# Autodesk Inventor assembly: Редуктор в сборе
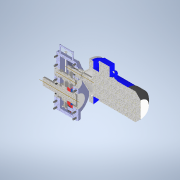
[picture p0: Inventor's stored thumbnail of the model, 180x180]
Saved by Autodesk Inventor 2021 (Build 250183000, 183)
## iProperties
Created: 2023-03-03
Part Number: Редуктор в сборе
Document SubType Name: Assembly
Designer: gdevc
Mass: 20906 g
Surface Area: 13580.9 cm^2
Volume: 12356.7 cm^3
Density: 1.69188 g/cm^3
Author: gdevc
## Documents named in this file (26)
- C:\Users\gdevc\OneDrive\Рабочий стол\Курсач\DetaliMashine\Новая папка\Редуктор в сборе.iam
- C:\Users\gdevc\OneDrive\Рабочий стол\Курсач\DetaliMashine\Новая папка\Вал_промежуточный.ipt
- C:\Users\gdevc\OneDrive\Рабочий стол\Курсач\DetaliMashine\Новая папка\Редуктор в сборе\Мастер проектирования\Цилиндрическое зубчатое зацепление1.iam
- C:\Users\gdevc\OneDrive\Рабочий стол\Курсач\DetaliMashine\Новая папка\Колесо быстроходное.ipt
- C:\Users\gdevc\OneDrive\Рабочий стол\Курсач\DetaliMashine\Новая папка\Редуктор в сборе\Мастер проектирования\Цилиндрическое зубчатое зацепление2.iam
- C:\Users\gdevc\OneDrive\Рабочий стол\Курсач\DetaliMashine\Новая папка\Вал_тихоходный.ipt
- C:\Users\gdevc\OneDrive\Рабочий стол\Курсач\DetaliMashine\Новая папка\Редуктор в сборе\Мастер проектирования\Цилиндрическое зубчатое зацепление3.iam
- C:\Users\gdevc\OneDrive\Рабочий стол\Курсач\DetaliMashine\Новая папка\Валл быстроходный.ipt
- C:\Users\gdevc\OneDrive\Рабочий стол\Курсач\DetaliMashine\Новая папка\Редуктор в сборе\Мастер проектирования\Цилиндрическое зубчатое зацепление4.iam
- C:\Users\gdevc\OneDrive\Рабочий стол\Курсач\DetaliMashine\Новая папка\Крышка тих_выход.ipt
- C:\Users\gdevc\OneDrive\Рабочий стол\Курсач\DetaliMashine\Новая папка\Крышка, тихая.ipt
- C:\Users\gdevc\OneDrive\Рабочий стол\Курсач\DetaliMashine\Новая папка\Крышка_пром.ipt
- C:\Users\gdevc\OneDrive\Рабочий стол\Курсач\DetaliMashine\Новая папка\Корпус.v.2.0.iam
- C:\Users\gdevc\OneDrive\Рабочий стол\Курсач\DetaliMashine\Новая папка\Манжет 1-30x47x7 ГОСТ 8752-79.ipt
- C:\Users\gdevc\OneDrive\Рабочий стол\Курсач\DetaliMashine\Новая папка\Крышка_быстроходного.ipt
- C:\Users\gdevc\OneDrive\Рабочий стол\Курсач\DetaliMashine\Новая папка\Подшипник 210 ГОСТ 8338-75.ipt
- C:\Users\gdevc\OneDrive\Рабочий стол\Курсач\DetaliMashine\Новая папка\Подшипник 205 ГОСТ 8338-75.ipt
- C:\Users\gdevc\OneDrive\Рабочий стол\Курсач\DetaliMashine\Новая папка\Манжет 2-50x65x8 ГОСТ 8752-79.ipt
- C:\Users\gdevc\OneDrive\Рабочий стол\Курсач\DetaliMashine\Новая папка\Болт M10×35 ГОСТ Р 50793-95.ipt
- C:\Users\gdevc\OneDrive\Рабочий стол\Курсач\DetaliMashine\Новая папка\Промежуточное колесо резина.ipt
- C:\Users\gdevc\OneDrive\Рабочий стол\Курсач\DetaliMashine\Новая папка\Редуктор в сборе\Мастер проектирования\Цилиндрическое зубчатое зацепление5.iam
- C:\Users\gdevc\OneDrive\Рабочий стол\Курсач\DetaliMashine\Новая папка\Резина конец.ipt
- C:\Users\gdevc\OneDrive\Рабочий стол\Курсач\DetaliMashine\Новая папка\Редуктор в сборе\Мастер проектирования\Цилиндрическое зубчатое зацепление6.iam
- C:\Users\gdevc\Downloads\Telegram Desktop\АИР100L IM2081 (2,4,6,8 пол)....ipt
- C:\Users\gdevc\OneDrive\Рабочий стол\Курсач\DetaliMashine\Новая папка\Редуктор в сборе\Мастер проектирования\Цилиндрическое зубчатое зацепление7.iam
- C:\Users\gdevc\OneDrive\Рабочий стол\Курсач\DetaliMashine\Новая папка\Шуп масло.ipt
## Components (36 placed, 19 different names)
1. Вал_промежуточный:1 — Совмещение:68, Совмещение:69, Совмещение:70
2. Цилиндрическое зубчатое зацепление:1 [sub-assembly]
3. Колесо быстроходное:1 — Заподлицо:3, Заподлицо:4, Заподлицо:7, Совмещение:69
4. Цилиндрическое зубчатое зацепление:2 [sub-assembly]
5. Вал_тихоходный:1 — Совмещение:10, Совмещение:11, Совмещение:12, Совмещение:13, Совмещение:18, Совмещение:21, Совмещение:23, Совмещение:29, Совмещение:55, Совмещение:58
6. Цилиндрическое зубчатое зацепление:3 [sub-assembly]
7. Валл быстроходный:1 — Заподлицо:3, Совмещение:32, Угол:3, Совмещение:36, Совмещение:56, Угол:4, Совмещение:67, Заподлицо:7
8. Цилиндрическое зубчатое зацепление:4 [sub-assembly]
9. Подшипник 205 ГОСТ 8338-75:1 — Совмещение:26, Совмещение:64
10. Подшипник 205 ГОСТ 8338-75:2 — Совмещение:28, Совмещение:66, Совмещение:70
11. Подшипник 210 ГОСТ 8338-75:1 — Совмещение:10, Совмещение:11
12. Подшипник 210 ГОСТ 8338-75:2 — Совмещение:12, Совмещение:13, Совмещение:30
13. Манжет 2-50x65x8 ГОСТ 8752-79:1 — Совмещение:18
14. Крышка тих_выход:1 — Совмещение:21, Совмещение:30, Совмещение:71
15. Крышка, тихая:1 — Совмещение:23, Совмещение:35
16. Крышка_пром:1 — Совмещение:26, Совмещение:63, Заподлицо:6, Совмещение:64, Совмещение:67, Совмещение:68
17. Крышка_пром:2 — Совмещение:28, Совмещение:31, Совмещение:65, Совмещение:66
18. Корпус.v.2.0:1 [sub-assembly] — Совмещение:29, Угол:2, Совмещение:31, Совмещение:34, Совмещение:35, Совмещение:37, Совмещение:38, Совмещение:39, Совмещение:40, Совмещение:41, Совмещение:42, Совмещение:43, Совмещение:44, Совмещение:45, Совмещение:46, Совмещение:47, Совмещение:48, Совмещение:49, Совмещение:50, Совмещение:51, Совмещение:52, Совмещение:53, Совмещение:54, Совмещение:59, Совмещение:61, Совмещение:62, Совмещение:63, Заподлицо:6, Совмещение:65, Совмещение:71
19. Манжет 1-30x47x7 ГОСТ 8752-79:1 — Совмещение:32, Совмещение:33
20. Крышка_быстроходного:1 — Совмещение:33, Совмещение:34, Совмещение:60
21. Болт M10×35 ГОСТ Р 50793-95:1 — Совмещение:37, Совмещение:46
22. Болт M10×35 ГОСТ Р 50793-95:2 — Совмещение:38, Совмещение:47
23. Болт M10×35 ГОСТ Р 50793-95:3 — Совмещение:39, Совмещение:49
24. Болт M10×35 ГОСТ Р 50793-95:4 — Совмещение:40, Совмещение:48
25. Болт M10×35 ГОСТ Р 50793-95:5 — Совмещение:41, Совмещение:51
26. Болт M10×35 ГОСТ Р 50793-95:6 — Совмещение:42, Совмещение:53
27. Болт M10×35 ГОСТ Р 50793-95:7 — Совмещение:43, Совмещение:50
28. Болт M10×35 ГОСТ Р 50793-95:8 — Совмещение:44, Совмещение:52
29. Болт M10×35 ГОСТ Р 50793-95:9 — Совмещение:45, Совмещение:54
30. Промежуточное колесо резина:1 — Совмещение:55, Заподлицо:4, Заподлицо:5
31. Цилиндрическое зубчатое зацепление:5 [sub-assembly]
32. Резина конец:1 — Совмещение:58, Совмещение:59, Заподлицо:5
33. Цилиндрическое зубчатое зацепление:6 [sub-assembly]
34. АИР100L IM2081 (2,4,6,8 пол)...:1 — Совмещение:56, Угол:4, Совмещение:60
35. Цилиндрическое зубчатое зацепление:7 [sub-assembly]
36. Шуп масло:1 — Совмещение:61, Совмещение:62
## Relationships (59: Mate 51, Flush 5, Angle 3)
- Совмещение:10 [Mate]: Вал_тихоходный:1 ↔ Подшипник 210 ГОСТ 8338-75:1
- Совмещение:11 [Mate]: Вал_тихоходный:1 ↔ Подшипник 210 ГОСТ 8338-75:1
- Совмещение:12 [Mate]: Вал_тихоходный:1 ↔ Подшипник 210 ГОСТ 8338-75:2
- Совмещение:13 [Mate]: Вал_тихоходный:1 ↔ Подшипник 210 ГОСТ 8338-75:2
- Совмещение:18 [Mate]: Вал_тихоходный:1 ↔ Манжет 2-50x65x8 ГОСТ 8752-79:1
- Совмещение:21 [Mate]: Вал_тихоходный:1 ↔ Крышка тих_выход:1
- Совмещение:23 [Mate]: Вал_тихоходный:1 ↔ Крышка, тихая:1
- Совмещение:26 [Mate]: Подшипник 205 ГОСТ 8338-75:1 ↔ Крышка_пром:1
- Совмещение:28 [Mate]: Подшипник 205 ГОСТ 8338-75:2 ↔ Крышка_пром:2
- Совмещение:29 [Mate]: Вал_тихоходный:1 ↔ Корпус.v.2.0:1
- Угол:2 [Angle] (90 deg): Корпус.v.2.0:1
- Совмещение:30 [Mate]: Подшипник 210 ГОСТ 8338-75:2 ↔ Крышка тих_выход:1
- Совмещение:31 [Mate]: Крышка_пром:2 ↔ Корпус.v.2.0:1
- Заподлицо:3 [Flush] (-1 mm): Колесо быстроходное:1 ↔ Валл быстроходный:1
- Совмещение:32 [Mate]: Валл быстроходный:1 ↔ Манжет 1-30x47x7 ГОСТ 8752-79:1
- Совмещение:33 [Mate]: Манжет 1-30x47x7 ГОСТ 8752-79:1 ↔ Крышка_быстроходного:1
- Совмещение:34 [Mate]: Корпус.v.2.0:1 ↔ Крышка_быстроходного:1
- Совмещение:35 [Mate]: Крышка, тихая:1 ↔ Корпус.v.2.0:1
- Угол:3 [Angle] (90 deg): Валл быстроходный:1
- Совмещение:36 [Mate]: Валл быстроходный:1
- Совмещение:37 [Mate]: Корпус.v.2.0:1 ↔ Болт M10×35 ГОСТ Р 50793-95:1
- Совмещение:38 [Mate]: Корпус.v.2.0:1 ↔ Болт M10×35 ГОСТ Р 50793-95:2
- Совмещение:39 [Mate]: Корпус.v.2.0:1 ↔ Болт M10×35 ГОСТ Р 50793-95:3
- Совмещение:40 [Mate]: Корпус.v.2.0:1 ↔ Болт M10×35 ГОСТ Р 50793-95:4
- Совмещение:41 [Mate]: Корпус.v.2.0:1 ↔ Болт M10×35 ГОСТ Р 50793-95:5
- Совмещение:42 [Mate]: Корпус.v.2.0:1 ↔ Болт M10×35 ГОСТ Р 50793-95:6
- Совмещение:43 [Mate]: Корпус.v.2.0:1 ↔ Болт M10×35 ГОСТ Р 50793-95:7
- Совмещение:44 [Mate]: Корпус.v.2.0:1 ↔ Болт M10×35 ГОСТ Р 50793-95:8
- Совмещение:45 [Mate]: Корпус.v.2.0:1 ↔ Болт M10×35 ГОСТ Р 50793-95:9
- Совмещение:46 [Mate]: Корпус.v.2.0:1 ↔ Болт M10×35 ГОСТ Р 50793-95:1
- Совмещение:47 [Mate]: Корпус.v.2.0:1 ↔ Болт M10×35 ГОСТ Р 50793-95:2
- Совмещение:48 [Mate]: Корпус.v.2.0:1 ↔ Болт M10×35 ГОСТ Р 50793-95:4
- Совмещение:49 [Mate]: Корпус.v.2.0:1 ↔ Болт M10×35 ГОСТ Р 50793-95:3
- Совмещение:50 [Mate]: Корпус.v.2.0:1 ↔ Болт M10×35 ГОСТ Р 50793-95:7
- Совмещение:51 [Mate]: Корпус.v.2.0:1 ↔ Болт M10×35 ГОСТ Р 50793-95:5
- Совмещение:52 [Mate]: Корпус.v.2.0:1 ↔ Болт M10×35 ГОСТ Р 50793-95:8
- Совмещение:53 [Mate]: Корпус.v.2.0:1 ↔ Болт M10×35 ГОСТ Р 50793-95:6
- Совмещение:54 [Mate]: Корпус.v.2.0:1 ↔ Болт M10×35 ГОСТ Р 50793-95:9
- Совмещение:55 [Mate]: Вал_тихоходный:1 ↔ Промежуточное колесо резина:1
- Заподлицо:4 [Flush] (-1 mm): Колесо быстроходное:1 ↔ Промежуточное колесо резина:1
- Совмещение:56 [Mate]: Валл быстроходный:1 ↔ АИР100L IM2081 (2,4,6,8 пол)...:1
- Совмещение:58 [Mate] (-70.35 mm): Вал_тихоходный:1 ↔ Резина конец:1
- Совмещение:59 [Mate]: Корпус.v.2.0:1 ↔ Резина конец:1
- Заподлицо:5 [Flush] (-1 mm): Промежуточное колесо резина:1 ↔ Резина конец:1
- Угол:4 [Angle] (0 deg): Валл быстроходный:1 ↔ АИР100L IM2081 (2,4,6,8 пол)...:1
- Совмещение:60 [Mate]: Крышка_быстроходного:1 ↔ АИР100L IM2081 (2,4,6,8 пол)...:1
- Совмещение:61 [Mate]: Корпус.v.2.0:1 ↔ Шуп масло:1
- Совмещение:62 [Mate]: Корпус.v.2.0:1 ↔ Шуп масло:1
- Совмещение:63 [Mate]: Крышка_пром:1 ↔ Корпус.v.2.0:1
- Заподлицо:6 [Flush]: Крышка_пром:1 ↔ Корпус.v.2.0:1
- Совмещение:64 [Mate]: Подшипник 205 ГОСТ 8338-75:1 ↔ Крышка_пром:1
- Совмещение:65 [Mate]: Крышка_пром:2 ↔ Корпус.v.2.0:1
- Совмещение:66 [Mate]: Подшипник 205 ГОСТ 8338-75:2 ↔ Крышка_пром:2
- Совмещение:67 [Mate]: Валл быстроходный:1 ↔ Крышка_пром:1
- Совмещение:68 [Mate]: Вал_промежуточный:1 ↔ Крышка_пром:1
- Заподлицо:7 [Flush] (-1 mm): Колесо быстроходное:1 ↔ Валл быстроходный:1
- Совмещение:69 [Mate]: Вал_промежуточный:1 ↔ Колесо быстроходное:1
- Совмещение:70 [Mate]: Вал_промежуточный:1 ↔ Подшипник 205 ГОСТ 8338-75:2
- Совмещение:71 [Mate]: Крышка тих_выход:1 ↔ Корпус.v.2.0:1
